# Autodesk Inventor assembly: GearMotor_Wheel_MIR
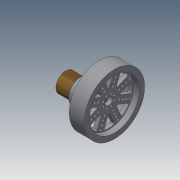
[picture p0: Inventor's stored thumbnail of the model, 180x180]
Saved by Autodesk Inventor 2014 SP1 (Build 180222100, 222)
## iProperties
Created: 2014-04-02
Part Number: GearMotor_Wheel_MIR
Document SubType Name: Assembly
Designer: tom
Author: tom
## Documents named in this file (5)
- C:\Users\tom\Documents\GitHub\Vacubot\Inventor\GearMotor_Wheel_MIR.iam
- C:\Users\tom\Documents\GitHub\Vacubot\Inventor\Motor Mount_MIR2.ipt
- C:\Users\tom\Documents\GitHub\Vacubot\Inventor\Drive Motor_MIR1.ipt
- C:\Users\tom\Documents\GitHub\Vacubot\Inventor\Clamping Hub_MIR.ipt
- C:\Users\tom\Documents\GitHub\Vacubot\Inventor\Wheel_MIR.ipt
## Components (4 placed, 4 different names)
1. Motor Mount_MIR2:1 — Flush:1, Mate:1
2. Drive Motor_MIR1:1 — Flush:1, Mate:1, Mate:3, Mate:2
3. Clamping Hub_MIR:1 — Mate:3, Mate:2, Mate:5, Mate:4
4. Wheel_MIR:1 — Mate:5, Mate:4
## Relationships (6: Mate 5, Flush 1)
- Flush:1 (-5 mm): Motor Mount_MIR2:1 ↔ Drive Motor_MIR1:1
- Mate:1: Motor Mount_MIR2:1 ↔ Drive Motor_MIR1:1
- Mate:3: Drive Motor_MIR1:1 ↔ Clamping Hub_MIR:1
- Mate:2: Drive Motor_MIR1:1 ↔ Clamping Hub_MIR:1
- Mate:5: Clamping Hub_MIR:1 ↔ Wheel_MIR:1
- Mate:4: Clamping Hub_MIR:1 ↔ Wheel_MIR:1
